# Autodesk Inventor assembly: thrust bearing_40mm
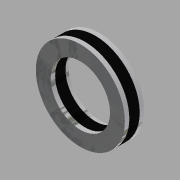
[picture p0: Inventor's stored thumbnail of the model, 180x180]
Saved by Autodesk Inventor 2019 (Build 230136000, 136)
## iProperties
Created: 2021-11-05
Part Number: thrust bearing_40mm
Document SubType Name: Assembly
Designer: Mohamed
Author: Mohamed
## Documents named in this file (4)
- F:\Semester 7\Design of mechatronics 1\SSCARA Robot\thrust bearing_40mm.iam
- F:\Semester 7\Design of mechatronics 1\SSCARA Robot\THRUST BEARING 40.ipt
- F:\Semester 7\Design of mechatronics 1\SSCARA Robot\thrust bearing 42.ipt
- F:\Semester 7\Design of mechatronics 1\SSCARA Robot\thrust bearing balls.ipt
## Components (3 placed, 3 different names)
1. THRUST BEARING 40:1 — Mate:3, Mate:4
2. thrust bearing 42:1 — Mate:1, Mate:2
3. thrust bearing balls:1 — Mate:1, Mate:2, Mate:3, Mate:4
## Relationships (4: Mate 4)
- Mate:1: thrust bearing 42:1 ↔ thrust bearing balls:1
- Mate:2: thrust bearing 42:1 ↔ thrust bearing balls:1
- Mate:3: THRUST BEARING 40:1 ↔ thrust bearing balls:1
- Mate:4: THRUST BEARING 40:1 ↔ thrust bearing balls:1
